# Autodesk Inventor assembly: Tank Tred_01
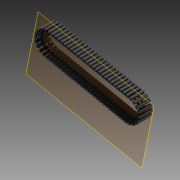
[picture p0: Inventor's stored thumbnail of the model, 180x180]
Saved by Autodesk Inventor 2013 (Build 170138000, 138)
## iProperties
Created: 2012-12-07
Part Number: Tank Tred_01
Document SubType Name: Assembly
Designer: zagerst
Author: zagerst
## Documents named in this file (2)
- \\lmss\STUDENTS\Robotics\CAD Files\4324 Robot - 2013\4324 Robot Omni-drive\Tank Treds\Tank Tred_01.iam
- \\lmss\STUDENTS\Robotics\CAD Files\4324 Robot - 2013\4324 Robot Omni-drive\Tank Treds\Tred Link.iam
## Components (70 placed, 1 different names)
1. Tred Link:1 [sub-assembly] — Insert:14, Insert:15, Flush:14, Flush:15
2. Tred Link:2 [sub-assembly] — Insert:31, Insert:32, Angle:6, Angle:7
3. Tred Link:3 [sub-assembly] — Insert:20, Insert:21, Flush:20, Flush:21
4. Tred Link:4 [sub-assembly] — Insert:16, Insert:17, Flush:16, Flush:17
5. Tred Link:5 [sub-assembly] — Insert:32, Insert:33, Angle:7, Angle:8
6. Tred Link:6 [sub-assembly] — Insert:29, Insert:30, Angle:4, Angle:5
7. Tred Link:7 [sub-assembly] — Insert:28, Insert:29, Angle:3, Angle:4
8. Tred Link:8 [sub-assembly] — Insert:26, Insert:27, Angle:1, Angle:2
9. Tred Link:9 [sub-assembly] — Insert:35, Insert:36, Angle:10, Flush:26
10. Tred Link:10 [sub-assembly] — Insert:36, Insert:37, Flush:26, Flush:27
11. Tred Link:11 [sub-assembly] — Insert:37, Insert:38, Flush:27, Flush:28
12. Tred Link:12 [sub-assembly] — Insert:38, Insert:39, Flush:28, Flush:29
13. Tred Link:13 [sub-assembly] — Insert:34, Insert:35, Angle:9
14. Tred Link:14 [sub-assembly] — Insert:33, Insert:34, Angle:8, Angle:9
15. Tred Link:15 [sub-assembly] — Insert:21, Insert:22, Flush:21, Flush:22
16. Tred Link:16 [sub-assembly] — Insert:18, Insert:19, Flush:18, Flush:19
17. Tred Link:17 [sub-assembly] — Insert:8, Insert:9, Flush:8, Flush:9
18. Tred Link:18 [sub-assembly] — Insert:11, Insert:12, Flush:11, Flush:12
19. Tred Link:19 [sub-assembly] — Insert:13, Insert:14, Flush:13, Flush:14
20. Tred Link:20 [sub-assembly] — Insert:23, Insert:24, Flush:23, Flush:24
21. Tred Link:21 [sub-assembly] — Insert:22, Insert:23, Flush:22, Flush:23
22. Tred Link:22 [sub-assembly] — Insert:30, Insert:31, Angle:5, Angle:6, Mate:1
23. Tred Link:23 [sub-assembly] — Insert:24, Insert:25, Flush:24, Flush:25, Angle:10
24. Tred Link:24 [sub-assembly] — Insert:25, Insert:26, Flush:25, Angle:1
25. Tred Link:25 [sub-assembly] — Insert:27, Insert:28, Angle:2, Angle:3
26. Tred Link:26 [sub-assembly] — Insert:12, Insert:13, Flush:12, Flush:13
27. Tred Link:27 [sub-assembly] — Insert:7, Insert:8, Flush:7, Flush:8
28. Tred Link:28 [sub-assembly] — Insert:5, Insert:6, Flush:5, Flush:6
29. Tred Link:29 [sub-assembly] — Insert:6, Insert:7, Flush:6, Flush:7
30. Tred Link:30 [sub-assembly] — Insert:1, Flush:1, Insert:59
31. Tred Link:31 [sub-assembly] — Insert:39, Flush:29, Insert:69, Flush:48
32. Tred Link:32 [sub-assembly] — Insert:1, Insert:2, Flush:1, Flush:2
33. Tred Link:33 [sub-assembly] — Insert:4, Insert:5, Flush:4, Flush:5
34. Tred Link:34 [sub-assembly] — Insert:3, Insert:4, Flush:3, Flush:4
35. Tred Link:35 [sub-assembly] — Insert:2, Insert:3, Flush:2, Flush:3
36. Tred Link:39 [sub-assembly] — Insert:15, Insert:16, Flush:15, Flush:16
37. Tred Link:40 [sub-assembly] — Insert:19, Insert:20, Flush:19, Flush:20
38. Tred Link:41 [sub-assembly] — Insert:17, Insert:18, Flush:17, Flush:18, Angle:21
39. Tred Link:42 [sub-assembly] — Insert:10, Insert:11, Flush:10, Flush:11
40. Tred Link:43 [sub-assembly] — Insert:9, Insert:10, Flush:9, Flush:10
41. Tred Link:44 [sub-assembly] — Insert:40, Flush:39, Insert:63, Flush:40
42. Tred Link:45 [sub-assembly] — Insert:45, Insert:46, Flush:33, Flush:34
43. Tred Link:46 [sub-assembly] — Insert:46, Insert:47, Flush:32, Flush:33
44. Tred Link:47 [sub-assembly] — Insert:48, Insert:49, Flush:30, Flush:31
45. Tred Link:48 [sub-assembly] — Insert:49, Insert:50, Flush:30, Angle:20
46. Tred Link:49 [sub-assembly] — Insert:50, Insert:51, Angle:19, Angle:20
47. Tred Link:50 [sub-assembly] — Insert:51, Insert:52, Angle:18, Angle:19
48. Tred Link:51 [sub-assembly] — Insert:52, Insert:53, Angle:17, Angle:18
49. Tred Link:52 [sub-assembly] — Insert:53, Insert:54, Angle:16, Angle:17
50. Tred Link:53 [sub-assembly] — Insert:54, Insert:55, Angle:15, Angle:16
51. Tred Link:54 [sub-assembly] — Insert:55, Insert:56, Angle:14, Angle:15
52. Tred Link:55 [sub-assembly] — Insert:40, Insert:41, Flush:38, Flush:39
53. Tred Link:56 [sub-assembly] — Insert:41, Insert:42, Flush:37, Flush:38
54. Tred Link:57 [sub-assembly] — Insert:42, Insert:43, Flush:36, Flush:37
55. Tred Link:58 [sub-assembly] — Insert:43, Insert:44, Flush:35, Flush:36
56. Tred Link:59 [sub-assembly] — Insert:57, Insert:58, Angle:12, Angle:13
57. Tred Link:60 [sub-assembly] — Insert:58, Insert:59, Angle:12
58. Tred Link:61 [sub-assembly] — Insert:56, Insert:57, Angle:13, Angle:14
59. Tred Link:62 [sub-assembly] — Insert:47, Insert:48, Flush:31, Flush:32
60. Tred Link:63 [sub-assembly] — Insert:44, Insert:45, Flush:34, Flush:35
61. Tred Link:64 [sub-assembly] — Insert:60, Flush:43, Insert:67, Flush:44
62. Tred Link:65 [sub-assembly] — Insert:60, Insert:61, Flush:42, Flush:43
63. Tred Link:66 [sub-assembly] — Insert:62, Insert:63, Flush:40, Flush:41
64. Tred Link:67 [sub-assembly] — Insert:64, Flush:47, Angle:21
65. Tred Link:68 [sub-assembly] — Insert:64, Insert:65, Flush:46, Flush:47
66. Tred Link:69 [sub-assembly] — Insert:66, Insert:67, Flush:44, Flush:45
67. Tred Link:70 [sub-assembly] — Insert:65, Insert:66, Flush:45, Flush:46
68. Tred Link:71 [sub-assembly] — Insert:61, Insert:62, Flush:41, Flush:42, Mate:2
69. Tred Link:72 [sub-assembly] — Insert:68, Flush:49
70. Tred Link:73 [sub-assembly] — Insert:68, Insert:69, Flush:48, Flush:49
## Relationships (140: Insert 69, Flush 49, Angle 20, Mate 2)
- Insert:1: Tred Link:30 ↔ Tred Link:32
- Insert:2: Tred Link:32 ↔ Tred Link:35
- Insert:3: Tred Link:34 ↔ Tred Link:35
- Insert:4: Tred Link:33 ↔ Tred Link:34
- Insert:5: Tred Link:28 ↔ Tred Link:33
- Insert:6: Tred Link:28 ↔ Tred Link:29
- Insert:7: Tred Link:27 ↔ Tred Link:29
- Insert:8: Tred Link:17 ↔ Tred Link:27
- Insert:9: Tred Link:17 ↔ Tred Link:43
- Insert:10: Tred Link:42 ↔ Tred Link:43
- Insert:11: Tred Link:18 ↔ Tred Link:42
- Insert:12: Tred Link:18 ↔ Tred Link:26
- Insert:13: Tred Link:19 ↔ Tred Link:26
- Insert:14: Tred Link:1 ↔ Tred Link:19
- Insert:15: Tred Link:1 ↔ Tred Link:39
- Insert:16: Tred Link:4 ↔ Tred Link:39
- Insert:17: Tred Link:4 ↔ Tred Link:41
- Insert:18: Tred Link:16 ↔ Tred Link:41
- Insert:19: Tred Link:16 ↔ Tred Link:40
- Insert:20: Tred Link:3 ↔ Tred Link:40
- Insert:21: Tred Link:3 ↔ Tred Link:15
- Insert:22: Tred Link:15 ↔ Tred Link:21
- Insert:23: Tred Link:20 ↔ Tred Link:21
- Insert:24: Tred Link:20 ↔ Tred Link:23
- Insert:25: Tred Link:23 ↔ Tred Link:24
- Insert:26: Tred Link:8 ↔ Tred Link:24
- Insert:27: Tred Link:8 ↔ Tred Link:25
- Insert:28: Tred Link:7 ↔ Tred Link:25
- Insert:29: Tred Link:6 ↔ Tred Link:7
- Insert:30: Tred Link:6 ↔ Tred Link:22
- Insert:31: Tred Link:2 ↔ Tred Link:22
- Insert:32: Tred Link:2 ↔ Tred Link:5
- Insert:33: Tred Link:5 ↔ Tred Link:14
- Insert:34: Tred Link:13 ↔ Tred Link:14
- Insert:35: Tred Link:9 ↔ Tred Link:13
- Insert:36: Tred Link:9 ↔ Tred Link:10
- Insert:37: Tred Link:10 ↔ Tred Link:11
- Insert:38: Tred Link:11 ↔ Tred Link:12
- Insert:39: Tred Link:12 ↔ Tred Link:31
- Flush:1: Tred Link:30 ↔ Tred Link:32
- Flush:2: Tred Link:32 ↔ Tred Link:35
- Flush:3: Tred Link:34 ↔ Tred Link:35
- Flush:4: Tred Link:33 ↔ Tred Link:34
- Flush:5: Tred Link:28 ↔ Tred Link:33
- Flush:6: Tred Link:28 ↔ Tred Link:29
- Flush:7: Tred Link:27 ↔ Tred Link:29
- Flush:8: Tred Link:17 ↔ Tred Link:27
- Flush:9: Tred Link:17 ↔ Tred Link:43
- Flush:10: Tred Link:42 ↔ Tred Link:43
- Flush:11: Tred Link:18 ↔ Tred Link:42
- Flush:12: Tred Link:18 ↔ Tred Link:26
- Flush:13: Tred Link:19 ↔ Tred Link:26
- Flush:14: Tred Link:1 ↔ Tred Link:19
- Flush:15: Tred Link:1 ↔ Tred Link:39
- Flush:16: Tred Link:4 ↔ Tred Link:39
- Flush:17: Tred Link:4 ↔ Tred Link:41
- Flush:18: Tred Link:16 ↔ Tred Link:41
- Flush:19: Tred Link:16 ↔ Tred Link:40
- Flush:20: Tred Link:3 ↔ Tred Link:40
- Flush:21: Tred Link:3 ↔ Tred Link:15
- Flush:22: Tred Link:15 ↔ Tred Link:21
- Flush:23: Tred Link:20 ↔ Tred Link:21
- Flush:24: Tred Link:20 ↔ Tred Link:23
- Flush:25: Tred Link:23 ↔ Tred Link:24
- Angle:1 (12.64 deg): Tred Link:8 ↔ Tred Link:24
- Angle:2 (19.56 deg): Tred Link:8 ↔ Tred Link:25
- Angle:3 (19.56 deg): Tred Link:7 ↔ Tred Link:25
- Angle:4 (19.56 deg): Tred Link:6 ↔ Tred Link:7
- Angle:5 (19.56 deg): Tred Link:6 ↔ Tred Link:22
- Angle:6 (19.56 deg): Tred Link:2 ↔ Tred Link:22
- Angle:7 (19.56 deg): Tred Link:2 ↔ Tred Link:5
- Angle:8 (19.56 deg): Tred Link:5 ↔ Tred Link:14
- Angle:9 (19.56 deg): Tred Link:13 ↔ Tred Link:14
- Angle:10 (180 deg): Tred Link:9 ↔ Tred Link:23
- Flush:26: Tred Link:9 ↔ Tred Link:10
- Flush:27: Tred Link:10 ↔ Tred Link:11
- Flush:28: Tred Link:11 ↔ Tred Link:12
- Flush:29: Tred Link:12 ↔ Tred Link:31
- Insert:40: Tred Link:44 ↔ Tred Link:55
- Insert:41: Tred Link:55 ↔ Tred Link:56
- Insert:42: Tred Link:56 ↔ Tred Link:57
- Insert:43: Tred Link:57 ↔ Tred Link:58
- Insert:44: Tred Link:58 ↔ Tred Link:63
- Insert:45: Tred Link:45 ↔ Tred Link:63
- Insert:46: Tred Link:45 ↔ Tred Link:46
- Insert:47: Tred Link:46 ↔ Tred Link:62
- Insert:48: Tred Link:47 ↔ Tred Link:62
- Insert:49: Tred Link:47 ↔ Tred Link:48
- Insert:50: Tred Link:48 ↔ Tred Link:49
- Insert:51: Tred Link:49 ↔ Tred Link:50
- Insert:52: Tred Link:50 ↔ Tred Link:51
- Insert:53: Tred Link:51 ↔ Tred Link:52
- Insert:54: Tred Link:52 ↔ Tred Link:53
- Insert:55: Tred Link:53 ↔ Tred Link:54
- Insert:56: Tred Link:54 ↔ Tred Link:61
- Insert:57: Tred Link:59 ↔ Tred Link:61
- Insert:58: Tred Link:59 ↔ Tred Link:60
- Insert:59: Tred Link:30 ↔ Tred Link:60
- Angle:12 (19.56 deg): Tred Link:59 ↔ Tred Link:60
- Angle:13 (-19.56 deg): Tred Link:59 ↔ Tred Link:61
- Angle:14 (-19.56 deg): Tred Link:54 ↔ Tred Link:61
- Angle:15 (-19.56 deg): Tred Link:53 ↔ Tred Link:54
- Angle:16 (-19.56 deg): Tred Link:52 ↔ Tred Link:53
- Angle:17 (-19.56 deg): Tred Link:51 ↔ Tred Link:52
- Angle:18 (-19.56 deg): Tred Link:50 ↔ Tred Link:51
- Angle:19 (-19.56 deg): Tred Link:49 ↔ Tred Link:50
- Flush:30: Tred Link:47 ↔ Tred Link:48
- Flush:31: Tred Link:47 ↔ Tred Link:62
- Flush:32: Tred Link:46 ↔ Tred Link:62
- Flush:33: Tred Link:45 ↔ Tred Link:46
- Flush:34: Tred Link:45 ↔ Tred Link:63
- Flush:35: Tred Link:58 ↔ Tred Link:63
- Flush:36: Tred Link:57 ↔ Tred Link:58
- Flush:37: Tred Link:56 ↔ Tred Link:57
- Flush:38: Tred Link:55 ↔ Tred Link:56
- Flush:39: Tred Link:44 ↔ Tred Link:55
- Insert:60: Tred Link:64 ↔ Tred Link:65
- Insert:61: Tred Link:65 ↔ Tred Link:71
- Insert:62: Tred Link:66 ↔ Tred Link:71
- Insert:63: Tred Link:44 ↔ Tred Link:66
- Flush:40: Tred Link:44 ↔ Tred Link:66
- Flush:41: Tred Link:66 ↔ Tred Link:71
- Flush:42: Tred Link:65 ↔ Tred Link:71
- Flush:43: Tred Link:64 ↔ Tred Link:65
- Insert:64: Tred Link:67 ↔ Tred Link:68
- Insert:65: Tred Link:68 ↔ Tred Link:70
- Insert:66: Tred Link:69 ↔ Tred Link:70
- Insert:67: Tred Link:64 ↔ Tred Link:69
- Flush:44: Tred Link:64 ↔ Tred Link:69
- Flush:45: Tred Link:69 ↔ Tred Link:70
- Flush:46: Tred Link:68 ↔ Tred Link:70
- Flush:47: Tred Link:67 ↔ Tred Link:68
- Insert:68: Tred Link:72 ↔ Tred Link:73
- Insert:69: Tred Link:31 ↔ Tred Link:73
- Flush:48: Tred Link:31 ↔ Tred Link:73
- Flush:49: Tred Link:72 ↔ Tred Link:73
- Angle:20 (12.56 deg): Tred Link:48 ↔ Tred Link:49
- Angle:21 (180 deg): Tred Link:41 ↔ Tred Link:67
- Mate:1: Tred Link:22
- Mate:2: Tred Link:71
